# Autodesk Inventor assembly: Сборка_крепления_динамика
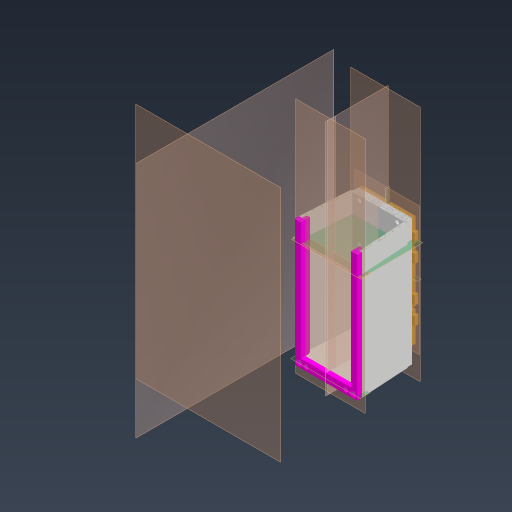
[picture p0: Inventor's stored thumbnail of the model, 512x512]
Saved by Autodesk Inventor 2023.2 (Build 272271030, 271C)
## iProperties
Created: 2025-09-18
Part Number: Сборка_крепления_динамика
Document SubType Name: Assembly
Designer: Олег Коноваленко
Author: Олег Коноваленко
## Documents named in this file (4)
- D:\!project\fox_n_crow_construction\crow\face\Сборка_крепления_динамика.iam
- D:\!project\fox_n_crow_construction\crow\face\Фанерка ерпления колонок.ipt
- D:\!project\fox_n_crow_construction\crow\face\Крепление_новой_колонки.ipt
- D:\!project\fox_n_crow_construction\crow\face\Проставка_крепления_ динамика.ipt
## Components (3 placed, 3 different names)
1. Фанерка ерпления колонок:1 — Совмещение:1, Совмещение:2, Заподлицо:1
2. Крепление_новой_колонки:1 — Совмещение:1, Совмещение:2, Заподлицо:1, Совмещение:3, Заподлицо:2
3. Проставка_крепления_ динамика:1 — Совмещение:3, Заподлицо:2
## Relationships (5: Mate 3, Flush 2)
- Совмещение:1 [Mate]: Фанерка ерпления колонок:1 ↔ Крепление_новой_колонки:1
- Совмещение:2 [Mate]: Фанерка ерпления колонок:1 ↔ Крепление_новой_колонки:1
- Заподлицо:1 [Flush]: Фанерка ерпления колонок:1 ↔ Крепление_новой_колонки:1
- Совмещение:3 [Mate]: Крепление_новой_колонки:1 ↔ Проставка_крепления_ динамика:1
- Заподлицо:2 [Flush]: Крепление_новой_колонки:1 ↔ Проставка_крепления_ динамика:1
